# Autodesk Inventor assembly: chainTest
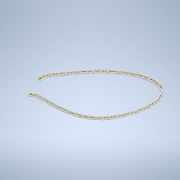
[picture p0: Inventor's stored thumbnail of the model, 180x180]
Saved by Autodesk Inventor 2020.3 (Build 243373000, 373)
## iProperties
Created: 2021-03-03
Part Number: chainTest
Document SubType Name: Assembly
Designer: con_c_000
Author: con_c_000
## Documents named in this file (3)
- C:\Users\con_c_000\Documents\Inventor\Content Center Files\FIRST ROBOT\chainTest.iam
- C:\Users\con_c_000\Documents\Inventor\Content Center Files\FIRST ROBOT\chainLink.ipt
- C:\Users\con_c_000\Documents\Inventor\Content Center Files\FIRST ROBOT\chainLink2.ipt
## Components (41 placed, 2 different names)
1. chainLink:1
2. chainLink2:1
3. chainLink2:2
4. chainLink2:3
5. chainLink2:4
6. chainLink2:5
7. chainLink2:6
8. chainLink2:7
9. chainLink2:8
10. chainLink2:9
11. chainLink2:10
12. chainLink2:11
13. chainLink2:12
14. chainLink2:13
15. chainLink2:14
16. chainLink2:15
17. chainLink2:16
18. chainLink2:17
19. chainLink2:18
20. chainLink2:19
21. chainLink2:20
22. chainLink2:21
23. chainLink2:22
24. chainLink2:23
25. chainLink2:24
26. chainLink2:25
27. chainLink2:26
28. chainLink2:27
29. chainLink2:28
30. chainLink2:29
31. chainLink2:30
32. chainLink2:31
33. chainLink2:32
34. chainLink2:33
35. chainLink2:34
36. chainLink2:35
37. chainLink2:36
38. chainLink2:37
39. chainLink2:38
40. chainLink2:39
41. chainLink2:40
## Relationships (40: Composite 40)
- [Composite]: chainLink:1 ↔ chainLink2:1
- [Composite]: chainLink2:1 ↔ chainLink2:2
- [Composite]: chainLink2:2 ↔ chainLink2:3
- [Composite]: chainLink2:3 ↔ chainLink2:4
- [Composite]: chainLink2:4 ↔ chainLink2:5
- [Composite]: chainLink2:5 ↔ chainLink2:6
- [Composite]: chainLink2:6 ↔ chainLink2:7
- [Composite]: chainLink2:7 ↔ chainLink2:8
- [Composite]: chainLink2:8 ↔ chainLink2:9
- [Composite]: chainLink2:9 ↔ chainLink2:10
- [Composite]: chainLink2:10 ↔ chainLink2:11
- [Composite]: chainLink2:11 ↔ chainLink2:12
- [Composite]: chainLink2:12 ↔ chainLink2:13
- [Composite]: chainLink2:13 ↔ chainLink2:14
- [Composite]: chainLink2:14 ↔ chainLink2:15
- [Composite]: chainLink2:15 ↔ chainLink2:16
- [Composite]: chainLink2:16 ↔ chainLink2:17
- [Composite]: chainLink2:17 ↔ chainLink2:18
- [Composite]: chainLink2:18 ↔ chainLink2:19
- [Composite]: chainLink2:19 ↔ chainLink2:20
- [Composite]: chainLink2:20 ↔ chainLink2:21
- [Composite]: chainLink2:21 ↔ chainLink2:22
- [Composite]: chainLink2:22 ↔ chainLink2:23
- [Composite]: chainLink2:23 ↔ chainLink2:24
- [Composite]: chainLink2:24 ↔ chainLink2:25
- [Composite]: chainLink2:25 ↔ chainLink2:26
- [Composite]: chainLink2:26 ↔ chainLink2:27
- [Composite]: chainLink2:27 ↔ chainLink2:28
- [Composite]: chainLink2:28 ↔ chainLink2:29
- [Composite]: chainLink2:29 ↔ chainLink2:30
- [Composite]: chainLink2:30 ↔ chainLink2:31
- [Composite]: chainLink2:31 ↔ chainLink2:32
- [Composite]: chainLink2:32 ↔ chainLink2:33
- [Composite]: chainLink2:33 ↔ chainLink2:34
- [Composite]: chainLink2:34 ↔ chainLink2:35
- [Composite]: chainLink2:35 ↔ chainLink2:36
- [Composite]: chainLink2:36 ↔ chainLink2:37
- [Composite]: chainLink2:37 ↔ chainLink2:38
- [Composite]: chainLink2:38 ↔ chainLink2:39
- [Composite]: chainLink2:39 ↔ chainLink2:40
